# Autodesk Inventor assembly: Electronics
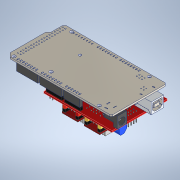
[picture p0: Inventor's stored thumbnail of the model, 180x180]
Saved by Autodesk Inventor 2022 (Build 260153000, 153)
## iProperties
Created: 2022-03-15
Part Number: Electronics
Document SubType Name: Assembly
Designer: JK
Author: JK
## Documents named in this file (3)
- C:\Users\JK\Documents\Inventor\ScaraNema\SCARA-3DP\Parts\Electronics\Electronics.iam
- C:\Users\JK\Documents\Inventor\ScaraNema\SCARA-3DP\Parts\Electronics\Arduino Mega 2560 v1.ipt
- C:\Users\JK\Documents\Inventor\ScaraNema\SCARA-3DP\Parts\Electronics\Arduino UNO and Shield\Arduino_Uno_CNC_Shield_V3.ipt
## Components (2 placed, 2 different names)
1. Arduino Mega 2560 v1:1 — Coincidencia:1, Nivelación:1, Nivelación:2
2. Arduino_Uno_CNC_Shield_V3:1 — Coincidencia:1, Nivelación:1, Nivelación:2
## Relationships (3: Flush 2, Mate 1)
- Coincidencia:1 [Mate]: Arduino Mega 2560 v1:1 ↔ Arduino_Uno_CNC_Shield_V3:1
- Nivelación:1 [Flush]: Arduino Mega 2560 v1:1 ↔ Arduino_Uno_CNC_Shield_V3:1
- Nivelación:2 [Flush]: Arduino Mega 2560 v1:1 ↔ Arduino_Uno_CNC_Shield_V3:1
